# Autodesk Inventor assembly: SMC_CJ1KB10-45
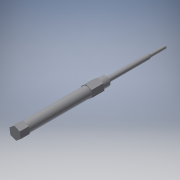
[picture p0: Inventor's stored thumbnail of the model, 180x180]
Saved by Autodesk Inventor 2018 (Build 220112000, 112)
## iProperties
Created: 2018-04-28
Part Number: SMC_CJ1KB10-45
Material: 一般
Document SubType Name: Assembly
Designer: Take
Author: Take
## Documents named in this file (3)
- C:\Users\Take\Documents\Inventor\パーツ\SMC_CJ1KB10-45.iam
- C:\Users\Take\Documents\Inventor\パーツ\SMC_CJ1KB10-45(本体).ipt
- C:\Users\Take\Documents\Inventor\パーツ\SMC_CJ1KB10-45(円柱).ipt
## Components (2 placed, 2 different names)
1. SMC_CJ1KB10-45(本体):1 — 円柱状:1, メイト:1
2. SMC_CJ1KB10-45(円柱):1 — 円柱状:1, メイト:1
## Relationships (2: CylindricalJoint 1, Mate 1)
- 円柱状:1 [CylindricalJoint]: SMC_CJ1KB10-45(本体):1 ↔ SMC_CJ1KB10-45(円柱):1
- メイト:1 [Mate]: SMC_CJ1KB10-45(本体):1 ↔ SMC_CJ1KB10-45(円柱):1
